# Autodesk Inventor assembly: RT_ELE_001_ElectricalMainPlate_V0.3
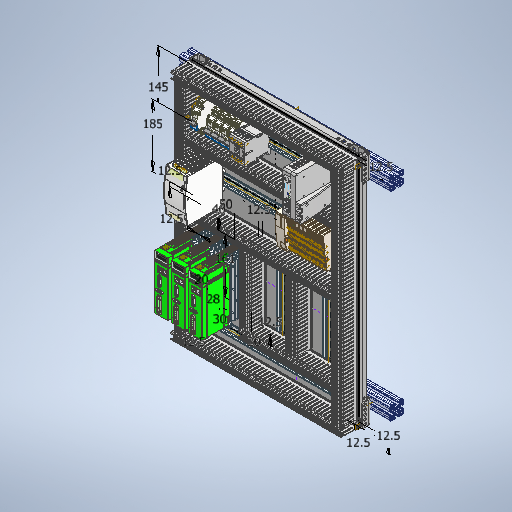
[picture p0: Inventor's stored thumbnail of the model, 512x512]
Saved by Autodesk Inventor 2025.4 (Build 294407000, 407)
## iProperties
Created: 2026-06-07
Part Number: RT_ELE_001_ElectricalMainPlate_V0.3
Document SubType Name: Assembly
Designer: louis
Author: louis
## Documents named in this file (18)
- C:\Users\louis\OneDrive\Desktop\R_Trident\02_CAD\04_Subassemblies\RT_ELE_001_ElectricalMainPlate_V0.3.iam
- C:\Users\louis\OneDrive\Desktop\R_Trident\02_CAD\01_Standard_Parts\04_ELE_Electrical_Automation\A6-400EC\A6-400EC.iam
- C:\Users\louis\OneDrive\Desktop\R_Trident\02_CAD\01_Standard_Parts\04_ELE_Electrical_Automation\VX 8617540\8617_540.iam
- C:\Users\louis\OneDrive\Desktop\R_Trident\02_CAD\01_Standard_Parts\04_ELE_Electrical_Automation\Cable channel 60x25\Cable channel 60x25x670.ipt
- C:\Users\louis\OneDrive\Desktop\R_Trident\02_CAD\01_Standard_Parts\04_ELE_Electrical_Automation\Cable channel 60x25\Cable channel 60x25x500.ipt
- C:\Users\louis\OneDrive\Desktop\R_Trident\02_CAD\01_Standard_Parts\04_ELE_Electrical_Automation\wdr_240_24\WDR-240-24.iam
- C:\Users\louis\OneDrive\Desktop\R_Trident\02_CAD\01_Standard_Parts\04_ELE_Electrical_Automation\Cable channel 60x25\Cable channel 60x25x430.ipt
- C:\Users\louis\OneDrive\Desktop\R_Trident\02_CAD\01_Standard_Parts\04_ELE_Electrical_Automation\WagoIO\Wago_IO_Module.iam
- C:\Users\louis\OneDrive\Desktop\R_Trident\02_CAD\04_Subassemblies\PI5_Case.iam
- C:\Users\louis\OneDrive\Desktop\R_Trident\02_CAD\01_Standard_Parts\04_ELE_Electrical_Automation\NFN 102\NCN006.ipt
- C:\Users\louis\OneDrive\Desktop\R_Trident\02_CAD\01_Standard_Parts\04_ELE_Electrical_Automation\NFN 102\NCN013.ipt
- C:\Users\louis\OneDrive\Desktop\R_Trident\02_CAD\01_Standard_Parts\04_ELE_Electrical_Automation\dilm7-10_24vdc_.ipt
- C:\Users\louis\OneDrive\Desktop\R_Trident\02_CAD\01_Standard_Parts\04_ELE_Electrical_Automation\WagoIO\280-519_LO.ipt
- C:\Users\louis\OneDrive\Desktop\R_Trident\02_CAD\01_Standard_Parts\04_ELE_Electrical_Automation\RT_DinRail_440.ipt
- C:\Users\louis\OneDrive\Desktop\R_Trident\02_CAD\01_Standard_Parts\04_ELE_Electrical_Automation\RT_DinRail_200.ipt
- C:\Users\louis\OneDrive\Desktop\R_Trident\02_CAD\01_Standard_Parts\04_ELE_Electrical_Automation\Cable channel 60x25\Cable channel 60x25x270.ipt
- C:\Users\louis\OneDrive\Desktop\R_Trident\02_CAD\01_Standard_Parts\04_ELE_Electrical_Automation\Cable channel 60x25\Cable channel 60x25x200.ipt
- C:\Users\louis\OneDrive\Desktop\R_Trident\02_CAD\01_Standard_Parts\02_FRM_Extrusions_Frame_V5\4040x620.ipt
## Components (30 placed, 17 different names)
1. 8617_540:1 [sub-assembly] — Flush:1, Flush:2, Flush:3, Mate:1, Mate:2, Mate:3, Mate:4, Mate:5, Mate:6, Mate:7, Mate:8, Mate:9, Mate:10, Mate:11, Mate:12, Mate:13, Mate:14, Mate:15, Mate:16, Mate:17, Mate:18, Mate:19, Mate:20, Mate:21, Mate:22, Mate:23, Mate:26, Mate:27, Mate:28, Mate:29, Mate:30, Mate:31, Mate:43, Mate:44, Mate:45, Mate:46, Mate:49, Mate:50, Mate:51, Mate:52, Mate:53, Mate:54, Mate:56, Mate:57, Mate:58, Mate:61, Mate:65, Mate:67, Mate:69
2. RT_DinRail_440:1 — Mate:2, Mate:9, Mate:24, Mate:25, Flush:4, Mate:34, Flush:5, Mate:35, Flush:6, Mate:36, Flush:7, Mate:37, Flush:8, Mate:38, Mate:39, Mate:40, Mate:41, Mate:42
3. RT_DinRail_440:2 — Mate:3, Mate:10
4. RT_DinRail_440:3 — Mate:1, Mate:11, Mate:32, Mate:33
5. A6-400EC:1 [sub-assembly] — Mate:4, Mate:14, Mate:15
6. A6-400EC:2 [sub-assembly] — Mate:5, Mate:16, Mate:17
7. A6-400EC:3 [sub-assembly] — Mate:6, Mate:18, Mate:19
8. Cable channel 60x25x670:1 — Mate:8, Mate:12
9. Cable channel 60x25x670:2 — Mate:7, Mate:13
10. Cable channel 60x25x500:1 — Mate:20, Mate:21
11. Cable channel 60x25x500:2 — Mate:22, Mate:23
12. WDR-240-24:1 [sub-assembly] — Mate:24, Mate:25, Mate:26
13. Cable channel 60x25x430:1 — Mate:27, Mate:28
14. Cable channel 60x25x430:2 — Mate:29, Mate:30
15. Wago_IO_Module:1 [sub-assembly] — Mate:31, Mate:32
16. PI5_Case:1 [sub-assembly] — Mate:33
17. NCN006:1 — Flush:4, Mate:34
18. NCN006:2 — Flush:5, Mate:35
19. NCN006:3 — Flush:6, Mate:36
20. NCN006:4 — Flush:7, Mate:37
21. NCN013:1 — Flush:8, Mate:38
22. dilm7-10_24vdc_:1 — Mate:39, Mate:40
23. 280-519_LO:1 — Mate:41, Mate:42
24. RT_DinRail_200:1 — Mate:43, Mate:44
25. RT_DinRail_200:2 — Mate:45, Mate:46
26. Cable channel 60x25x200:1 — Mate:49, Mate:50
27. Cable channel 60x25x270:1 — Mate:51, Mate:52
28. Cable channel 60x25x200:2 — Mate:53, Mate:54
29. 4040x620:1 — Mate:64, Mate:65, Mate:68, Mate:69
30. 4040x620:2 — Mate:66, Mate:67, Mate:68
## Relationships (74: Mate 66, Flush 8)
- Flush:1: 8617_540:1
- Flush:2: 8617_540:1
- Flush:3: 8617_540:1
- Mate:1: 8617_540:1 ↔ RT_DinRail_440:3
- Mate:2: 8617_540:1 ↔ RT_DinRail_440:1
- Mate:3: 8617_540:1 ↔ RT_DinRail_440:2
- Mate:4: 8617_540:1 ↔ A6-400EC:1
- Mate:5: 8617_540:1 ↔ A6-400EC:2
- Mate:6: 8617_540:1 ↔ A6-400EC:3
- Mate:7: 8617_540:1 ↔ Cable channel 60x25x670:2
- Mate:8: 8617_540:1 ↔ Cable channel 60x25x670:1
- Mate:9: 8617_540:1 ↔ RT_DinRail_440:1
- Mate:10: 8617_540:1 ↔ RT_DinRail_440:2
- Mate:11: 8617_540:1 ↔ RT_DinRail_440:3
- Mate:12: 8617_540:1 ↔ Cable channel 60x25x670:1
- Mate:13: 8617_540:1 ↔ Cable channel 60x25x670:2
- Mate:14: 8617_540:1 ↔ A6-400EC:1
- Mate:15: 8617_540:1 ↔ A6-400EC:1
- Mate:16: 8617_540:1 ↔ A6-400EC:2
- Mate:17: 8617_540:1 ↔ A6-400EC:2
- Mate:18: 8617_540:1 ↔ A6-400EC:3
- Mate:19: 8617_540:1 ↔ A6-400EC:3
- Mate:20: 8617_540:1 ↔ Cable channel 60x25x500:1
- Mate:21: 8617_540:1 ↔ Cable channel 60x25x500:1
- Mate:22: 8617_540:1 ↔ Cable channel 60x25x500:2
- Mate:23: 8617_540:1 ↔ Cable channel 60x25x500:2
- Mate:24: RT_DinRail_440:1 ↔ WDR-240-24:1
- Mate:25: RT_DinRail_440:1 ↔ WDR-240-24:1
- Mate:26: 8617_540:1 ↔ WDR-240-24:1
- Mate:27: 8617_540:1 ↔ Cable channel 60x25x430:1
- Mate:28: 8617_540:1 ↔ Cable channel 60x25x430:1
- Mate:29: 8617_540:1 ↔ Cable channel 60x25x430:2
- Mate:30: 8617_540:1 ↔ Cable channel 60x25x430:2
- Mate:31: 8617_540:1 ↔ Wago_IO_Module:1
- Mate:32: RT_DinRail_440:3 ↔ Wago_IO_Module:1
- Mate:33: RT_DinRail_440:3 ↔ PI5_Case:1
- Flush:4: RT_DinRail_440:1 ↔ NCN006:1
- Mate:34: RT_DinRail_440:1 ↔ NCN006:1
- Flush:5: RT_DinRail_440:1 ↔ NCN006:2
- Mate:35: RT_DinRail_440:1 ↔ NCN006:2
- Flush:6: RT_DinRail_440:1 ↔ NCN006:3
- Mate:36: RT_DinRail_440:1 ↔ NCN006:3
- Flush:7: RT_DinRail_440:1 ↔ NCN006:4
- Mate:37: RT_DinRail_440:1 ↔ NCN006:4
- Flush:8: RT_DinRail_440:1 ↔ NCN013:1
- Mate:38: RT_DinRail_440:1 ↔ NCN013:1
- Mate:39: RT_DinRail_440:1 ↔ dilm7-10_24vdc_:1
- Mate:40: RT_DinRail_440:1 ↔ dilm7-10_24vdc_:1
- Mate:41: RT_DinRail_440:1 ↔ 280-519_LO:1
- Mate:42: RT_DinRail_440:1 ↔ 280-519_LO:1
- Mate:43: 8617_540:1 ↔ RT_DinRail_200:1
- Mate:44: 8617_540:1 ↔ RT_DinRail_200:1
- Mate:45: 8617_540:1 ↔ RT_DinRail_200:2
- Mate:46: 8617_540:1 ↔ RT_DinRail_200:2
- Mate:49: 8617_540:1 ↔ Cable channel 60x25x200:1
- Mate:50: 8617_540:1 ↔ Cable channel 60x25x200:1
- Mate:51: 8617_540:1 ↔ Cable channel 60x25x270:1
- Mate:52: 8617_540:1 ↔ Cable channel 60x25x270:1
- Mate:53: 8617_540:1 ↔ Cable channel 60x25x200:2
- Mate:54: 8617_540:1 ↔ Cable channel 60x25x200:2
- Mate:56: 8617_540:1
- Mate:57: 8617_540:1
- Mate:58: 8617_540:1
- Mate:59
- Mate:60
- Mate:61: 8617_540:1
- Mate:62
- Mate:63
- Mate:64: 4040x620:1
- Mate:65: 8617_540:1 ↔ 4040x620:1
- Mate:66: 4040x620:2
- Mate:67: 8617_540:1 ↔ 4040x620:2
- Mate:68: 4040x620:1 ↔ 4040x620:2
- Mate:69: 8617_540:1 ↔ 4040x620:1
